# Autodesk Inventor assembly: extension_assembly
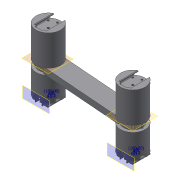
[picture p0: Inventor's stored thumbnail of the model, 180x180]
Saved by Autodesk Inventor 2018 (Build 220112000, 112)
## iProperties
Created: 2018-08-17
Part Number: extension_assembly
Document SubType Name: Assembly
Designer: Bardo91
Author: Bardo91
## Documents named in this file (3)
- E:\programming\hecatonquiros\cad_models\arm_4_dof\serial_model\extension_assembly.iam
- E:\programming\hecatonquiros\cad_models\arm_4_dof\serial_model\arm_0_extension.ipt
- E:\programming\hecatonquiros\cad_models\arm_4_dof\serial_model\arm_0_extension_attacher.ipt
## Components (3 placed, 2 different names)
1. arm_0_extension:1 — Mate:1, Mate:3
2. arm_0_extension:2 — Mate:2
3. arm_0_extension_attacher:1 — Mate:1, Mate:2, Mate:3
## Relationships (3: Mate 3)
- Mate:1: arm_0_extension:1 ↔ arm_0_extension_attacher:1
- Mate:2: arm_0_extension:2 ↔ arm_0_extension_attacher:1
- Mate:3: arm_0_extension:1 ↔ arm_0_extension_attacher:1
